# Autodesk Inventor assembly: Assembly1
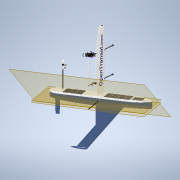
[picture p0: Inventor's stored thumbnail of the model, 180x180]
Saved by Autodesk Inventor 2020 (Build 240168000, 168)
## iProperties
Created: 2016-11-10
Part Number: Assembly1
Document SubType Name: Assembly
Designer: jous
Mass: 132842 g
Surface Area: 67379.5 cm^2
Volume: 131941 cm^3
Density: 1.00683 g/cm^3
Author: jous
## Documents named in this file (18)
- C:\Users\jous\Desktop\boat\boat.iam
- C:\Users\jous\Desktop\boat\hull.ipt
- C:\Users\jous\Desktop\boat\solar1.ipt
- C:\Users\jous\Desktop\boat\solar2.ipt
- C:\Users\jous\Desktop\boat\hatch.ipt
- C:\Users\jous\Desktop\boat\anemo.ipt
- C:\Users\jous\Desktop\boat\H4FM_2528_21.ipt
- C:\Users\jous\Desktop\boat\washer4.ipt
- C:\Users\jous\Desktop\boat\camera.ipt
- C:\Users\jous\Desktop\boat\battery_tube.iam
- C:\Users\jous\Desktop\boat\solar3.ipt
- C:\Users\jous\Desktop\boat\hall_sensor.ipt
- C:\Users\jous\Desktop\boat\text.ipt
- C:\Users\jous\Desktop\boat\LED.ipt
- C:\Users\jous\Desktop\boat\housing.ipt
- C:\Users\jous\Desktop\boat\skeleton.iam
- C:\Users\jous\Desktop\boat\sail.iam
- C:\Users\jous\Desktop\boat\keel.iam
## Components (22 placed, 17 different names)
1. hull:1 — Mate:1, Mate:2, Mate:9, Mate:11, Mate:13, Mate:14, Mate:15, Mate:16
2. skeleton:1 [sub-assembly] — Cylindrical:1, Rotational:9, Rotational:12, Rigid:1
3. hatch:1 — Mate:2
4. hatch:2 — Mate:1
5. anemo:1 — Rotational:6, Cylindrical:1
6. H4FM_2528_21:1 — Rotational:2, Rotational:12
7. washer4:1 — Rotational:2, Rotational:11
8. H4FM_2528_21:2 — Rotational:5, Rotational:9
9. washer4:2 — Rotational:5
10. camera:1 — Rotational:6
11. battery_tube:2 [sub-assembly]
12. battery_tube:3 [sub-assembly]
13. solar3:1 — Mate:16
14. solar1:1 — Mate:15
15. solar2:1 — Mate:14
16. hall_sensor:1 — Mate:9
17. text:1 — Mate:11
18. LED:1 — Mate:13
19. housing:1
20. housing:2
21. sail:1 [sub-assembly] — Rotational:11
22. keel:2 [sub-assembly] — Rigid:1
## Relationships (16: Mate 8, RevoluteJoint 6, CylindricalJoint 1, WeldJoint 1)
- Mate:1: hull:1 ↔ hatch:2
- Mate:2: hull:1 ↔ hatch:1
- Rotational:2 [RevoluteJoint]: H4FM_2528_21:1 ↔ washer4:1
- Rotational:5 [RevoluteJoint]: H4FM_2528_21:2 ↔ washer4:2
- Rotational:6 [RevoluteJoint] (-37.25 mm): anemo:1 ↔ camera:1
- Mate:9: hull:1 ↔ hall_sensor:1
- Mate:11: hull:1 ↔ text:1
- Mate:13: hull:1 ↔ LED:1
- Mate:14: hull:1 ↔ solar2:1
- Mate:15: hull:1 ↔ solar1:1
- Mate:16: hull:1 ↔ solar3:1
- Cylindrical:1: skeleton:1 ↔ anemo:1
- Rotational:9 [RevoluteJoint]: skeleton:1 ↔ H4FM_2528_21:2
- Rotational:11 [RevoluteJoint]: washer4:1 ↔ sail:1
- Rotational:12 [RevoluteJoint]: skeleton:1 ↔ H4FM_2528_21:1
- Rigid:1 [WeldJoint] (-250 mm): skeleton:1 ↔ keel:2
